# Autodesk Inventor assembly: Assembly_SIMMO_2
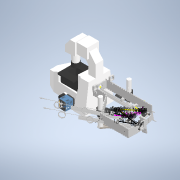
[picture p0: Inventor's stored thumbnail of the model, 180x180]
Saved by Autodesk Inventor 2022 (Build 260153000, 153)
## iProperties
Created: 2022-04-09
Part Number: Assembly_SIMMO_2
Document SubType Name: Assembly
Designer: Prakash Lab
Author: Prakash Lab
## Documents named in this file (28)
- C:\Users\diederichbenedict\Dropbox\Dokumente\Promotion\PROJECTS\SIMMO\INVENTOR\Assembly_SIMMO_1.iam
- C:\Users\diederichbenedict\Dropbox\Dokumente\Promotion\PROJECTS\SIMMO\INVENTOR\00_AC254-200-A-ML-Step.ipt
- C:\Users\diederichbenedict\Dropbox\Dokumente\Promotion\PROJECTS\SIMMO\INVENTOR\Adapter_DMD_KM100.ipt
- C:\Users\diederichbenedict\Dropbox\Dokumente\Promotion\PROJECTS\SIMMO\INVENTOR\Cover_new.ipt
- C:\Users\diederichbenedict\Dropbox\Dokumente\Promotion\PROJECTS\SIMMO\INVENTOR\KM100-Solidworks.ipt
- C:\Users\diederichbenedict\Dropbox\Dokumente\Promotion\PROJECTS\SIMMO\INVENTOR\Mount_new.ipt
- C:\Users\diederichbenedict\Dropbox\Dokumente\Promotion\PROJECTS\SIMMO\INVENTOR\Nikon_Ti2E.ipt
- C:\Users\diederichbenedict\Dropbox\Dokumente\Promotion\PROJECTS\SIMMO\INVENTOR\00_AC254-030-A-ML-Step.ipt
- C:\Users\diederichbenedict\Dropbox\Dokumente\Promotion\PROJECTS\SIMMO\INVENTOR\00_AC254-075-A-ML-Step.ipt
- C:\Users\diederichbenedict\Dropbox\Dokumente\Promotion\PROJECTS\SIMMO\INVENTOR\00_Beampath_v0.ipt
- C:\Users\diederichbenedict\Dropbox\Dokumente\Promotion\PROJECTS\SIMMO\INVENTOR\00_Assembly_Axiovert.ipt
- C:\Users\diederichbenedict\Dropbox\Dokumente\Promotion\PROJECTS\SIMMO\INVENTOR\00_KM100-Step.ipt
- C:\Users\diederichbenedict\Dropbox\Dokumente\Promotion\PROJECTS\SIMMO\INVENTOR\00_P1-305A-FC-1-Step.ipt
- C:\Users\diederichbenedict\Dropbox\Dokumente\Promotion\PROJECTS\SIMMO\INVENTOR\00_PF10-03-P01-Solidworks.ipt
- C:\Users\diederichbenedict\Dropbox\Dokumente\Promotion\PROJECTS\SIMMO\INVENTOR\00_Baseplate_Simmo_base.ipt
- C:\Users\diederichbenedict\Dropbox\Dokumente\Promotion\PROJECTS\SIMMO\INVENTOR\00_B3060L-Step.ipt
- C:\Users\diederichbenedict\Dropbox\Dokumente\Promotion\PROJECTS\SIMMO\INVENTOR\Assembly_Post_v0.iam
- C:\Users\diederichbenedict\Dropbox\Dokumente\Promotion\PROJECTS\SIMMO\INVENTOR\00_PCO_edge-det.ipt
- C:\Users\diederichbenedict\Dropbox\Dokumente\Promotion\PROJECTS\SIMMO\INVENTOR\00_Baseplate_Simmo_side1.ipt
- C:\Users\diederichbenedict\Dropbox\Dokumente\Promotion\PROJECTS\SIMMO\INVENTOR\00_Baseplate_Simmo_side3.ipt
- C:\Users\diederichbenedict\Dropbox\Dokumente\Promotion\PROJECTS\SIMMO\INVENTOR\00_Baseplate_Simmo_side2.ipt
- C:\Users\diederichbenedict\Dropbox\Dokumente\Promotion\PROJECTS\SIMMO\INVENTOR\00_Baseplate_Simmo_side4.ipt
- C:\Users\diederichbenedict\Dropbox\Dokumente\Promotion\PROJECTS\SIMMO\INVENTOR\00_Aluminium_Extrusion_20x20.ipt
- C:\Users\diederichbenedict\Dropbox\Dokumente\Promotion\PROJECTS\SIMMO\INVENTOR\10_Mountinplate_Mirrors_v0.ipt
- C:\Users\diederichbenedict\Dropbox\Dokumente\Promotion\PROJECTS\SIMMO\INVENTOR\00_Baseplate_Simmo_side5.ipt
- C:\Users\diederichbenedict\Dropbox\Dokumente\Promotion\PROJECTS\SIMMO\INVENTOR\00_Baseplate_Simmo_side6.ipt
- C:\Users\diederichbenedict\Dropbox\Dokumente\Promotion\PROJECTS\SIMMO\INVENTOR\00_Baseplate_Simmo_top.ipt
- C:\Users\diederichbenedict\Dropbox\Dokumente\Promotion\PROJECTS\SIMMO\INVENTOR\RailOptiX-Base-6-2_ThorlabsAC254.ipt
## Components (46 placed, 26 different names)
1. Adapter_DMD_KM100:1 — Insert:5, Mate:5, Insert:6, Mate:6
2. KM100-Solidworks:1 — Insert:6, Angle:3, Einfügen:35, Winkel:12
3. Mount_new:1 — Mate:6
4. Nikon_Ti2E:1 — Mate:1, Mate:2, Mate:3, Flush:1, Flush:2, Flush:4, Mate:10, Mate:11, Angle:6, Fluchtend:7, Fluchtend:8, Passend:25, Passend:26, Passend:32, Passend:33
5. 00_Beampath_v0:1 — Flush:1, Flush:2, Insert:1, Insert:3, Angle:1, Mate:12, Insert:23, Insert:25, Insert:27, Insert:29, Passend:29, Passend:33, Passend:36
6. 00_AC254-200-A-ML-Step:1 — Insert:1
7. 00_AC254-075-A-ML-Step:2 — Insert:3
8. Cover_new:1 — Angle:1, Angle:2, Insert:5, Mate:5
9. 00_Assembly_Axiovert:1 — Flush:4, Mate:10, Mate:11, Mate:12, Passend:13, Insert:36
10. 00_KM100-Step:2 — Insert:16, Angle:8, Einfügen:33, Winkel:10
11. 00_P1-305A-FC-1-Step:1 — Insert:28
12. 00_KM100-Step:3 — Insert:14, Angle:6, Einfügen:34, Winkel:11
13. 00_PF10-03-P01-Solidworks:1 — Insert:14
14. 00_PF10-03-P01-Solidworks:2 — Insert:16, Insert:23
15. 00_Baseplate_Simmo_side1:1
16. 00_KM100-Step:5 — Insert:21, Angle:9, Fluchtend:17, Fluchtend:18
17. 00_PF10-03-P01-Solidworks:3 — Insert:21, Insert:25
18. 00_P1-305A-FC-1-Step:2 — Insert:26
19. 00_AC254-030-A-ML-Step:2 — Insert:26, Insert:27
20. 00_Baseplate_Simmo_side3:1 — Passend:20, Fluchtend:14, Passend:21
21. 00_Baseplate_Simmo_side2 — Flush:15
22. 00_Baseplate_Simmo_side4:1 — Passend:22, Fluchtend:16, Fluchtend:22
23. 00_Aluminium_Extrusion_20x20:1 — Passend:24, Passend:25, Passend:26, Passend:40, Passend:41
24. 00_AC254-030-A-ML-Step:3 — Insert:28, Insert:29
25. 00_Baseplate_Simmo_base:1 — Fluchtend:7, Fluchtend:8, Angle:8, Angle:9, Passend:20, Fluchtend:14, Passend:21, Flush:15, Passend:22, Fluchtend:16, Passend:24, Fluchtend:19, Fluchtend:20, Passend:27, Fluchtend:21, Passend:30, Passend:35, Passend:37
26. 10_Mountinplate_Mirrors_v0:1 — Fluchtend:17, Fluchtend:18
27. 10_Mountinplate_Mirrors_v0:2 — Einfügen:33, Winkel:10
28. 10_Mountinplate_Mirrors_v0:3 — Einfügen:34, Winkel:11
29. 10_Mountinplate_Mirrors_v0:4 — Einfügen:35, Winkel:12
30. 00_Baseplate_Simmo_side2:2 — Fluchtend:19, Fluchtend:20, Passend:27, Fluchtend:23
31. 00_Baseplate_Simmo_side5:1 — Fluchtend:21
32. 00_Aluminium_Extrusion_20x20:2 — Passend:29, Passend:30, Passend:35
33. 00_AC254-075-A-ML-Step:3 — Passend:32
34. 00_Aluminium_Extrusion_20x20:3 — Passend:36, Passend:37
35. Assembly_Post_v0:2 [sub-assembly] — Passend:38
36. Assembly_Post_v0:3 [sub-assembly] — Passend:39
37. 00_Baseplate_Simmo_top:1 — Fluchtend:22, Fluchtend:23
38. 00_PCO_edge-det:2 — Insert:36
39. RailOptiX-Base-6-2_ThorlabsAC254:1 — Passend:40, Passend:41
40. RailOptiX-Base-6-2_ThorlabsAC254:2
41. RailOptiX-Base-6-2_ThorlabsAC254:3
42. RailOptiX-Base-6-2_ThorlabsAC254:4
43. 00_B3060L-Step:1 — Passend:13, Passend:38
44. 00_B3060L-Step:2 — Passend:39
45. 00_B3060L-Step:3
46. 00_B3060L-Step:4
## Component patterns: (4 elements, first: 00_B3060L-Step:1)
## Relationships (68: Mate 27, Insert 17, Flush 15, Angle 9)
- Mate:1: Nikon_Ti2E:1
- Mate:2: Nikon_Ti2E:1
- Mate:3: Nikon_Ti2E:1
- Flush:1: Nikon_Ti2E:1 ↔ 00_Beampath_v0:1
- Flush:2: Nikon_Ti2E:1 ↔ 00_Beampath_v0:1
- Insert:1: 00_Beampath_v0:1 ↔ 00_AC254-200-A-ML-Step:1
- Insert:3: 00_Beampath_v0:1 ↔ 00_AC254-075-A-ML-Step:2
- Angle:1 (190 deg): 00_Beampath_v0:1 ↔ Cover_new:1
- Angle:2 (0 deg): Cover_new:1
- Insert:5 (5 mm): Adapter_DMD_KM100:1 ↔ Cover_new:1
- Mate:5: Adapter_DMD_KM100:1 ↔ Cover_new:1
- Insert:6 (8 mm): Adapter_DMD_KM100:1 ↔ KM100-Solidworks:1
- Mate:6 (20 mm): Adapter_DMD_KM100:1 ↔ Mount_new:1
- Angle:3 (0 deg): KM100-Solidworks:1
- Flush:4: Nikon_Ti2E:1 ↔ 00_Assembly_Axiovert:1
- Mate:10: Nikon_Ti2E:1 ↔ 00_Assembly_Axiovert:1
- Mate:11: Nikon_Ti2E:1 ↔ 00_Assembly_Axiovert:1
- Mate:12 (-194 mm): 00_Beampath_v0:1 ↔ 00_Assembly_Axiovert:1
- Insert:14: 00_KM100-Step:3 ↔ 00_PF10-03-P01-Solidworks:1
- Angle:6 (0 deg): Nikon_Ti2E:1 ↔ 00_KM100-Step:3
- Insert:16: 00_KM100-Step:2 ↔ 00_PF10-03-P01-Solidworks:2
- Fluchtend:7 [Flush]: Nikon_Ti2E:1 ↔ 00_Baseplate_Simmo_base:1
- Fluchtend:8 [Flush]: Nikon_Ti2E:1 ↔ 00_Baseplate_Simmo_base:1
- Passend:13 [Mate]: 00_Assembly_Axiovert:1 ↔ 00_B3060L-Step:1
- Insert:21: 00_KM100-Step:5 ↔ 00_PF10-03-P01-Solidworks:3
- Insert:23: 00_Beampath_v0:1 ↔ 00_PF10-03-P01-Solidworks:2
- Insert:25: 00_Beampath_v0:1 ↔ 00_PF10-03-P01-Solidworks:3
- Insert:26 (50 mm): 00_P1-305A-FC-1-Step:2 ↔ 00_AC254-030-A-ML-Step:2
- Insert:27: 00_Beampath_v0:1 ↔ 00_AC254-030-A-ML-Step:2
- Angle:8 (180 deg): 00_KM100-Step:2 ↔ 00_Baseplate_Simmo_base:1
- Angle:9 (180 deg): 00_KM100-Step:5 ↔ 00_Baseplate_Simmo_base:1
- Passend:20 [Mate]: 00_Baseplate_Simmo_side3:1 ↔ 00_Baseplate_Simmo_base:1
- Fluchtend:14 [Flush]: 00_Baseplate_Simmo_side3:1 ↔ 00_Baseplate_Simmo_base:1
- Passend:21 [Mate] (0.1 mm): 00_Baseplate_Simmo_side3:1 ↔ 00_Baseplate_Simmo_base:1
- Flush:15: 00_Baseplate_Simmo_side2 ↔ 00_Baseplate_Simmo_base:1
- Passend:22 [Mate]: 00_Baseplate_Simmo_side4:1 ↔ 00_Baseplate_Simmo_base:1
- Fluchtend:16 [Flush]: 00_Baseplate_Simmo_side4:1 ↔ 00_Baseplate_Simmo_base:1
- Passend:24 [Mate]: 00_Aluminium_Extrusion_20x20:1 ↔ 00_Baseplate_Simmo_base:1
- Passend:25 [Mate]: Nikon_Ti2E:1 ↔ 00_Aluminium_Extrusion_20x20:1
- Passend:26 [Mate]: Nikon_Ti2E:1 ↔ 00_Aluminium_Extrusion_20x20:1
- Insert:28 (-50 mm): 00_P1-305A-FC-1-Step:1 ↔ 00_AC254-030-A-ML-Step:3
- Insert:29: 00_Beampath_v0:1 ↔ 00_AC254-030-A-ML-Step:3
- Fluchtend:17 [Flush]: 00_KM100-Step:5 ↔ 10_Mountinplate_Mirrors_v0:1
- Fluchtend:18 [Flush]: 00_KM100-Step:5 ↔ 10_Mountinplate_Mirrors_v0:1
- Einfügen:33 [Insert]: 00_KM100-Step:2 ↔ 10_Mountinplate_Mirrors_v0:2
- Winkel:10 [Angle] (0 deg): 00_KM100-Step:2 ↔ 10_Mountinplate_Mirrors_v0:2
- Einfügen:34 [Insert]: 00_KM100-Step:3 ↔ 10_Mountinplate_Mirrors_v0:3
- Winkel:11 [Angle] (0 deg): 00_KM100-Step:3 ↔ 10_Mountinplate_Mirrors_v0:3
- Einfügen:35 [Insert]: KM100-Solidworks:1 ↔ 10_Mountinplate_Mirrors_v0:4
- Winkel:12 [Angle] (0 deg): KM100-Solidworks:1 ↔ 10_Mountinplate_Mirrors_v0:4
- Fluchtend:19 [Flush]: 00_Baseplate_Simmo_base:1 ↔ 00_Baseplate_Simmo_side2:2
- Fluchtend:20 [Flush]: 00_Baseplate_Simmo_base:1 ↔ 00_Baseplate_Simmo_side2:2
- Passend:27 [Mate] (0.2 mm): 00_Baseplate_Simmo_base:1 ↔ 00_Baseplate_Simmo_side2:2
- Fluchtend:21 [Flush]: 00_Baseplate_Simmo_base:1 ↔ 00_Baseplate_Simmo_side5:1
- Passend:29 [Mate]: 00_Beampath_v0:1 ↔ 00_Aluminium_Extrusion_20x20:2
- Passend:30 [Mate]: 00_Baseplate_Simmo_base:1 ↔ 00_Aluminium_Extrusion_20x20:2
- Passend:32 [Mate]: Nikon_Ti2E:1 ↔ 00_AC254-075-A-ML-Step:3
- Passend:33 [Mate]: Nikon_Ti2E:1 ↔ 00_Beampath_v0:1
- Passend:35 [Mate]: 00_Baseplate_Simmo_base:1 ↔ 00_Aluminium_Extrusion_20x20:2
- Passend:36 [Mate]: 00_Beampath_v0:1 ↔ 00_Aluminium_Extrusion_20x20:3
- Passend:37 [Mate]: 00_Baseplate_Simmo_base:1 ↔ 00_Aluminium_Extrusion_20x20:3
- Passend:38 [Mate]: Assembly_Post_v0:2 ↔ 00_B3060L-Step:1
- Fluchtend:22 [Flush]: 00_Baseplate_Simmo_side4:1 ↔ 00_Baseplate_Simmo_top:1
- Fluchtend:23 [Flush]: 00_Baseplate_Simmo_side2:2 ↔ 00_Baseplate_Simmo_top:1
- Passend:39 [Mate]: Assembly_Post_v0:3 ↔ 00_B3060L-Step:2
- Insert:36: 00_Assembly_Axiovert:1 ↔ 00_PCO_edge-det:2
- Passend:40 [Mate]: 00_Aluminium_Extrusion_20x20:1 ↔ RailOptiX-Base-6-2_ThorlabsAC254:1
- Passend:41 [Mate]: 00_Aluminium_Extrusion_20x20:1 ↔ RailOptiX-Base-6-2_ThorlabsAC254:1
